# Autodesk Inventor assembly: Multi_Op_Setup
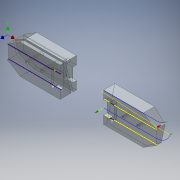
[picture p0: Inventor's stored thumbnail of the model, 180x180]
Saved by Autodesk Inventor 2018.3 (Build 223284000, 284)
## iProperties
Created: 2018-10-26
Part Number: Multi_Op_Setup
Project: =<Part Number>
Document SubType Name: Assembly
Designer: R.B.
Mass: 11681.1 g
Surface Area: 1929.13 cm^2
Volume: 1496.48 cm^3
Density: 7.80573 g/cm^3
Author: R.B.
## Documents named in this file (2)
- R:\CAD\~Aquafil~\7407 - 456 Slant Blades-72 Flat Blades (Standard Size)\CAD\Multi_Op_Setup.iam
- R:\CAD\~Aquafil~\7407 - 456 Slant Blades-72 Flat Blades (Standard Size)\CAD\DHC-1500-FF-02-003.ipt
## Components (3 placed, 1 different names)
1. DHC-1500-FF-02-003:1 — Flush:1, Flush:2, Flush:3, Flush:4, Mate:2, Mate:3
2. DHC-1500-FF-02-003:2 — Flush:1, Flush:2, Mate:3
3. DHC-1500-FF-02-003:3 — Flush:3, Flush:4, Mate:2
## Relationships (6: Flush 4, Mate 2)
- Flush:1: DHC-1500-FF-02-003:1 ↔ DHC-1500-FF-02-003:2
- Flush:2 (0.254 mm): DHC-1500-FF-02-003:1 ↔ DHC-1500-FF-02-003:2
- Flush:3: DHC-1500-FF-02-003:1 ↔ DHC-1500-FF-02-003:3
- Flush:4: DHC-1500-FF-02-003:1 ↔ DHC-1500-FF-02-003:3
- Mate:2 (-44.069 mm): DHC-1500-FF-02-003:1 ↔ DHC-1500-FF-02-003:3
- Mate:3 (-397.4846 mm): DHC-1500-FF-02-003:1 ↔ DHC-1500-FF-02-003:2
